# Autodesk Inventor assembly: FullAssembly
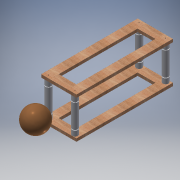
[picture p0: Inventor's stored thumbnail of the model, 180x180]
Saved by Autodesk Inventor 2016 (Build 200138000, 138)
## iProperties
Created: 2016-01-18
Part Number: FullAssembly
Document SubType Name: Assembly
Designer: yash
Author: yash
## Documents named in this file (4)
- C:\Users\yash\Documents\GitHub\Robotics2016\CAD\LowGoal\PickupPrototype0\FullAssembly.iam
- C:\Users\yash\Documents\GitHub\Robotics2016\CAD\LowGoal\PickupPrototype0\SingleSide.iam
- C:\Users\yash\Documents\GitHub\Robotics2016\CAD\LowGoal\PickupPrototype0\SpacerPiece.ipt
- C:\Users\yash\Documents\GitHub\Robotics2016\CAD\LowGoal\PickupPrototype0\Ball.ipt
## Components (7 placed, 3 different names)
1. SingleSide:1 [sub-assembly] — Mate:1, Mate:2, Mate:3, Mate:5, Mate:10, Mate:12, Mate:13, Mate:16, Mate:18, Mate:19, Mate:22, Mate:24
2. SpacerPiece:1 — Mate:1, Mate:2, Mate:3, Mate:4, Mate:7, Mate:8
3. SingleSide:2 [sub-assembly] — Mate:4, Mate:6, Mate:7, Mate:8, Mate:9, Mate:11, Mate:14, Mate:15, Mate:17, Mate:20, Mate:21, Mate:23, Mate:25
4. SpacerPiece:2 — Mate:5, Mate:6, Mate:9, Mate:10, Mate:11, Mate:12
5. SpacerPiece:3 — Mate:15, Mate:16, Mate:17, Mate:18, Mate:21, Mate:22, Mate:23
6. SpacerPiece:4 — Mate:13, Mate:14, Mate:19, Mate:20, Mate:24, Mate:25
7. Ball:1
## Relationships (25: Mate 25)
- Mate:1: SingleSide:1 ↔ SpacerPiece:1
- Mate:2: SingleSide:1 ↔ SpacerPiece:1
- Mate:3: SingleSide:1 ↔ SpacerPiece:1
- Mate:4: SpacerPiece:1 ↔ SingleSide:2
- Mate:5: SingleSide:1 ↔ SpacerPiece:2
- Mate:6: SingleSide:2 ↔ SpacerPiece:2
- Mate:7: SpacerPiece:1 ↔ SingleSide:2
- Mate:8: SpacerPiece:1 ↔ SingleSide:2
- Mate:9: SingleSide:2 ↔ SpacerPiece:2
- Mate:10: SingleSide:1 ↔ SpacerPiece:2
- Mate:11: SingleSide:2 ↔ SpacerPiece:2
- Mate:12: SingleSide:1 ↔ SpacerPiece:2
- Mate:13: SingleSide:1 ↔ SpacerPiece:4
- Mate:14: SingleSide:2 ↔ SpacerPiece:4
- Mate:15: SingleSide:2 ↔ SpacerPiece:3
- Mate:16: SingleSide:1 ↔ SpacerPiece:3
- Mate:17: SingleSide:2 ↔ SpacerPiece:3
- Mate:18: SingleSide:1 ↔ SpacerPiece:3
- Mate:19: SingleSide:1 ↔ SpacerPiece:4
- Mate:20: SingleSide:2 ↔ SpacerPiece:4
- Mate:21: SingleSide:2 ↔ SpacerPiece:3
- Mate:22: SingleSide:1 ↔ SpacerPiece:3
- Mate:23: SingleSide:2 ↔ SpacerPiece:3
- Mate:24: SingleSide:1 ↔ SpacerPiece:4
- Mate:25: SingleSide:2 ↔ SpacerPiece:4
